# Autodesk Inventor assembly: Full_Assembly
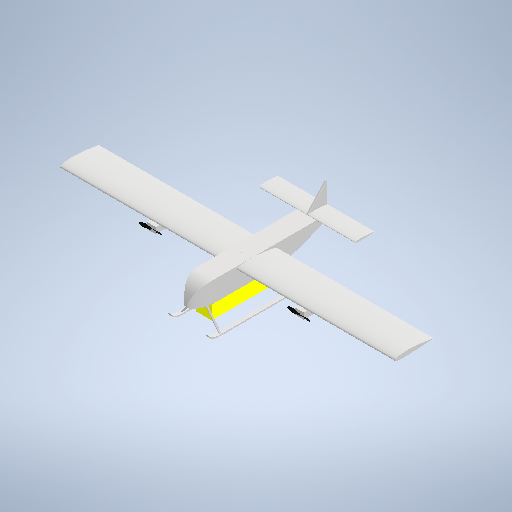
[picture p0: Inventor's stored thumbnail of the model, 512x512]
Saved by Autodesk Inventor 2027.1 (Build 311270010, 270A)
## iProperties
Created: 2026-09-09
Part Number: Full_Assembly
Document SubType Name: Assembly
Designer: PWYNNE
Author: PWYNNE
## Documents named in this file (17)
- C:\Users\pwynne\Desktop\GITHUB\SWIFT-UAV\System_development\Heron\structural_model\v0.1.0\Full_Assembly.iam
- C:\Users\pwynne\Desktop\GITHUB\SWIFT-UAV\System_development\Heron\structural_model\v0.1.0\fuselage.ipt
- C:\Users\pwynne\Desktop\GITHUB\SWIFT-UAV\System_development\Heron\structural_model\v0.1.0\Wing.ipt
- C:\Users\pwynne\Desktop\GITHUB\SWIFT-UAV\System_development\Heron\structural_model\v0.1.0\Wing_horizontal.ipt
- C:\Users\pwynne\Desktop\GITHUB\SWIFT-UAV\System_development\Heron\structural_model\v0.1.0\Wing_vertical.ipt
- C:\Users\pwynne\Desktop\GITHUB\SWIFT-UAV\System_development\Heron\structural_model\v0.1.0\Max_Payload.ipt
- C:\Users\pwynne\Desktop\GITHUB\SWIFT-UAV\System_development\Heron\structural_model\v0.1.0\Wing_MIR1.ipt
- C:\Users\pwynne\Desktop\GITHUB\SWIFT-UAV\System_development\Heron\structural_model\v0.1.0\Wing_horizontal_MIR3.ipt
- C:\Users\pwynne\Desktop\GITHUB\SWIFT-UAV\System_development\Heron\structural_model\v0.1.0\Landing_Skid.ipt
- C:\Users\pwynne\Desktop\GITHUB\SWIFT-UAV\System_development\Heron\structural_model\v0.1.0\Landing_Legs.ipt
- C:\Users\pwynne\Desktop\GITHUB\SWIFT-UAV\System_development\Heron\structural_model\v0.1.0\Forward_Motor.ipt
- C:\Users\pwynne\Desktop\GITHUB\SWIFT-UAV\System_development\Heron\structural_model\v0.1.0\Prop.ipt
- C:\Users\pwynne\Desktop\GITHUB\SWIFT-UAV\System_development\Heron\structural_model\v0.1.0\Forward_Motor_MIR.ipt
- C:\Users\pwynne\Desktop\GITHUB\SWIFT-UAV\System_development\Heron\structural_model\v0.1.0\Prop_MIR.ipt
- C:\Users\pwynne\Desktop\GITHUB\SWIFT-UAV\System_development\Heron\structural_model\v0.1.0\Prop_MIR1.ipt
- C:\Users\pwynne\Desktop\GITHUB\SWIFT-UAV\System_development\Heron\structural_model\v0.1.0\Landing_Legs_MIR3.ipt
- C:\Users\pwynne\Desktop\GITHUB\SWIFT-UAV\System_development\Heron\structural_model\v0.1.0\Landing_Skid_MIR2.ipt
## Components (17 placed, 16 different names)
1. fuselage:1 — Flush:2, Flush:3, Flush:5, Mate:3, Mate:5, Mate:6, Mate:7, Mate:9, Flush:12, Mate:10, Flush:13, Mate:11, Mate:12, Flush:15, Flush:19, Flush:20, Flush:21
2. Wing:1 — Mate:2, Mate:3, Mate:12
3. Wing_horizontal:1 — Mate:5, Mate:6, Flush:9, Mate:11
4. Wing_vertical:1 — Mate:7, Flush:9, Flush:13
5. Max_Payload:1 — Mate:9, Flush:12, Mate:10, Mate:13, Flush:16
6. Wing_MIR1:1 — Flush:14
7. Wing_horizontal_MIR3:1
8. Landing_Skid:1 — Mate:13, Mate:14, Flush:16, Flush:17, Mate:16, Mate:17
9. Landing_Legs:1 — Flush:17, Mate:16, Mate:17
10. Forward_Motor:1 — Flush:19, Flush:20, Flush:21, Flush:22, Flush:23, Mate:23
11. Prop:1 — Mate:21, Mate:22, Mate:23
12. Forward_Motor_MIR:1 — Flush:24, Flush:25
13. Prop_MIR:1
14. Prop_MIR1:1
15. Prop:2
16. Landing_Legs_MIR3:1
17. Landing_Skid_MIR2:1 — Mate:24
## Relationships (35: Flush 18, Mate 17)
- Flush:2 (-80 mm): fuselage:1
- Flush:3 (150 mm): fuselage:1
- Flush:4 (-1000 mm)
- Flush:5 (-250 mm): fuselage:1
- Mate:2: Wing:1
- Mate:3: fuselage:1 ↔ Wing:1
- Mate:5 (-60 mm): fuselage:1 ↔ Wing_horizontal:1
- Mate:6: fuselage:1 ↔ Wing_horizontal:1
- Mate:7: fuselage:1 ↔ Wing_vertical:1
- Flush:9: Wing_horizontal:1 ↔ Wing_vertical:1
- Mate:9: fuselage:1 ↔ Max_Payload:1
- Flush:12 (-10 mm): fuselage:1 ↔ Max_Payload:1
- Mate:10: fuselage:1 ↔ Max_Payload:1
- Flush:13: fuselage:1 ↔ Wing_vertical:1
- Mate:11: fuselage:1 ↔ Wing_horizontal:1
- Mate:12: fuselage:1 ↔ Wing:1
- Flush:14: Wing_MIR1:1
- Mate:13 (30 mm): Max_Payload:1 ↔ Landing_Skid:1
- Flush:15: fuselage:1
- Mate:14 (130 mm): Landing_Skid:1
- Flush:16 (-10 mm): Max_Payload:1 ↔ Landing_Skid:1
- Flush:17: Landing_Skid:1 ↔ Landing_Legs:1
- Mate:16 (-15 mm): Landing_Skid:1 ↔ Landing_Legs:1
- Mate:17 (12.5 mm): Landing_Skid:1 ↔ Landing_Legs:1
- Flush:19: fuselage:1 ↔ Forward_Motor:1
- Flush:20: fuselage:1 ↔ Forward_Motor:1
- Flush:21 (500 mm): fuselage:1 ↔ Forward_Motor:1
- Flush:22 (-35 mm): Forward_Motor:1
- Flush:23 (-23.89 mm): Forward_Motor:1
- Mate:21: Prop:1
- Mate:22: Prop:1
- Flush:24 (-35 mm): Forward_Motor_MIR:1
- Flush:25 (-23.89 mm): Forward_Motor_MIR:1
- Mate:23: Forward_Motor:1 ↔ Prop:1
- Mate:24 (130 mm): Landing_Skid_MIR2:1
